# Autodesk Inventor assembly: Почти готово_CPY
(part 2 of 2)
- Жесткий:6 [WeldJoint]: Палец_CPY:1 ↔ Стопорное кольцо_CPY:2
- Жесткий:16 [WeldJoint] (-5 mm): Втулка_CPY:1 ↔ Крышка цилиндра 1_CPY:1
- Жесткий:70 [WeldJoint] (-2 mm): Фонарь_CPY:1 ↔ Крышка цилиндра 2_CPY:1
- Жесткий:79 [WeldJoint]: Крышка цилиндра 2_CPY:1 ↔ Цилиндр2_CPY:1
- Жесткий:23 [WeldJoint] (1 mm): Крышка стакана_CPY:1 ↔ Цилиндр2_CPY:1
- Жесткий:15 [WeldJoint]: Втулка_CPY:1 ↔ Цилиндр2_CPY:1
- Жесткий:18 [WeldJoint]: Цилиндр2_CPY:1 ↔ Прокладка клапана_CPY:1
- Жесткий:81 [WeldJoint] (-22 mm): Цилиндр2_CPY:1 ↔ Стакан1_CPY:1
- Жесткий:61 [WeldJoint] (2 mm): Крышка цилиндра 2_CPY:1 ↔ Уплотнительное кольцо_CPY:1
- Жесткий:69 [WeldJoint]: Фонарь_CPY:1 ↔ Уплотнение фонарь_CPY:1
- Жесткий:95 [WeldJoint]: Корпус сальника перегородка 1_CPY:1 ↔ Крышка перегородки11_CPY:1
- Жесткий:94 [WeldJoint]: Фонарь_CPY:1 ↔ Крышка перегородки11_CPY:1
- Жесткий:96 [WeldJoint]: Корпус сальника перегородка 1_CPY:1 ↔ Крышка перегородки12_CPY:1
- Жесткий:104 [WeldJoint]: Корпус маслосъемника_CPY:1 ↔ Крышка перегородки21_CPY:1
- Жесткий:98 [WeldJoint]: Фонарь_CPY:1 ↔ Крышка перегородки21_CPY:1
- Жесткий:105 [WeldJoint]: Крышка перегородки21_CPY:1 ↔ Крышка перегородки22_CPY:1
- Жесткий:97 [WeldJoint]: Фонарь_CPY:1 ↔ Придав перегородки1_CPY:1
- Жесткий:106 [WeldJoint]: Фонарь_CPY:1 ↔ Придав перегородки1_CPY:2
- Жесткий:112 [WeldJoint]: Крышка цилиндра 1_CPY:1 ↔ Шайба  ГОСТ 11371-78 25:1
- Жесткий:113 [WeldJoint] (-8.75 mm): Шпилька ГОСТ 22038-76 M24-6g×70:1 ↔ Гайка ГОСТ 15524-70 M24:1
- Жесткий:111 [WeldJoint]: Цилиндр2_CPY:1 ↔ Шпилька ГОСТ 22038-76 M24-6g×70:1
- Жесткий:114 [WeldJoint] (-8.75 mm): Шпилька ГОСТ 22038-76 M24-6g×70:2 ↔ Гайка ГОСТ 15524-70 M24:2
- Жесткий:115 [WeldJoint]: Цилиндр2_CPY:1 ↔ Прокладка клапана_CPY:2
- Жесткий:117 [WeldJoint] (-22 mm): Цилиндр2_CPY:1 ↔ Стакан1_CPY:2
- Жесткий:118 [WeldJoint] (1 mm): Цилиндр2_CPY:1 ↔ Крышка стакана_CPY:2
- Жесткий:119 [WeldJoint] (-1 mm): Цилиндр2_CPY:1 ↔ Шпилька ГОСТ 22034-76 M20-6g×50:1
- Жесткий:121 [WeldJoint] (-5.5 mm): Гайка ГОСТ 15521-70 M20:1 ↔ Шпилька ГОСТ 22034-76 M20-6g×50:1
- Жесткий:120 [WeldJoint] (-23 mm): Шпилька ГОСТ 22034-76 M20-6g×50:1 ↔ Шайба ГОСТ 10450-78 19:1
- Жесткий:122 [WeldJoint] (1 mm): Цилиндр2_CPY:1 ↔ Шпилька ГОСТ 22034-76 M20-6g×50:2
- Жесткий:124 [WeldJoint] (-6.25 mm): Шпилька ГОСТ 22034-76 M20-6g×50:2 ↔ Гайка ГОСТ 15521-70 M20:2
- Жесткий:123 [WeldJoint] (-24 mm): Шпилька ГОСТ 22034-76 M20-6g×50:2 ↔ Шайба ГОСТ 10450-78 19:2
- Жесткий:127 [WeldJoint] (-2 mm): Фонарь_CPY:1 ↔ Гайка ГОСТ 15524-70 M20:1
- Жесткий:126 [WeldJoint] (-32 mm): Шпилька ГОСТ 22038-76 M20-6g×70:1 ↔ Шайба ГОСТ 10450-78 21:1
- Жесткий:125 [WeldJoint]: Крышка цилиндра 2_CPY:1 ↔ Шпилька ГОСТ 22038-76 M20-6g×70:1
- Жесткий:130 [WeldJoint]: Крышка перегородки22_CPY:1 ↔ Шайба  ГОСТ 11371-78 13:2
- Жесткий:134 [WeldJoint]: Придав перегородки1_CPY:1 ↔ Шайба  ГОСТ 11371-78 13:4
- Жесткий:128 [WeldJoint]: Крышка перегородки12_CPY:1 ↔ Шайба  ГОСТ 11371-78 13:1
- Жесткий:135 [WeldJoint]: Шайба  ГОСТ 11371-78 13:4 ↔ Винт ГОСТ 11738-84 M 10x25:2
- Жесткий:133 [WeldJoint]: Винт ГОСТ 11738-84 M 10x25:1 ↔ Шайба  ГОСТ 11371-78 13:3
- Жесткий:132 [WeldJoint]: Придав перегородки1_CPY:2 ↔ Шайба  ГОСТ 11371-78 13:3
- Жесткий:129 [WeldJoint]: Винт ГОСТ 11738-84 M 10x35:1 ↔ Шайба  ГОСТ 11371-78 13:1
- Жесткий:131 [WeldJoint]: Винт ГОСТ 11738-84 M 10x30:1 ↔ Шайба  ГОСТ 11371-78 13:2
- Жесткий:138 [WeldJoint] (-38 mm): Шпилька ГОСТ 22038-76 M24-6g×80:1 ↔ Гайка ГОСТ 15524-70 M24:18
- Жесткий:137 [WeldJoint] (-38 mm): Шпилька ГОСТ 22038-76 M24-6g×80:1 ↔ Шайба  ГОСТ 11371-78 28:1
- Жесткий:140 [WeldJoint] (-38 mm): Шпилька ГОСТ 22038-76 M24-6g×80:2 ↔ Гайка ГОСТ 15524-70 M24:19
- Жесткий:139 [WeldJoint] (-38 mm): Шпилька ГОСТ 22038-76 M24-6g×80:2 ↔ Шайба  ГОСТ 11371-78 28:2
- Жесткий:142 [WeldJoint] (-38 mm): Шпилька ГОСТ 22038-76 M24-6g×80:3 ↔ Гайка ГОСТ 15524-70 M24:20
- Жесткий:165 [WeldJoint]: Фонарь_CPY:1 ↔ Шайба  ГОСТ 11371-78 28:3
- Жесткий:141 [WeldJoint] (-38 mm): Шпилька ГОСТ 22038-76 M24-6g×80:3 ↔ Шайба  ГОСТ 11371-78 28:3
- Жесткий:144 [WeldJoint] (-38 mm): Шпилька ГОСТ 22038-76 M24-6g×80:4 ↔ Гайка ГОСТ 15524-70 M24:21
- Жесткий:166 [WeldJoint]: Фонарь_CPY:1 ↔ Шайба  ГОСТ 11371-78 28:4
- Жесткий:143 [WeldJoint] (-38 mm): Шпилька ГОСТ 22038-76 M24-6g×80:4 ↔ Шайба  ГОСТ 11371-78 28:4
- Жесткий:146 [WeldJoint] (-38 mm): Шпилька ГОСТ 22038-76 M24-6g×80:5 ↔ Гайка ГОСТ 15524-70 M24:22
- Жесткий:164 [WeldJoint]: Фонарь_CPY:1 ↔ Шайба  ГОСТ 11371-78 28:5
- Жесткий:145 [WeldJoint] (-38 mm): Шпилька ГОСТ 22038-76 M24-6g×80:5 ↔ Шайба  ГОСТ 11371-78 28:5
- Жесткий:148 [WeldJoint] (-38 mm): Шпилька ГОСТ 22038-76 M24-6g×80:6 ↔ Гайка ГОСТ 15524-70 M24:23
- Жесткий:171 [WeldJoint]: Фонарь_CPY:1 ↔ Шайба  ГОСТ 11371-78 28:6
- Жесткий:147 [WeldJoint] (-38 mm): Шпилька ГОСТ 22038-76 M24-6g×80:6 ↔ Шайба  ГОСТ 11371-78 28:6
- Жесткий:150 [WeldJoint] (-38 mm): Шпилька ГОСТ 22038-76 M24-6g×80:7 ↔ Гайка ГОСТ 15524-70 M24:24
- Жесткий:173 [WeldJoint]: Фонарь_CPY:1 ↔ Шайба  ГОСТ 11371-78 28:7
- Жесткий:149 [WeldJoint] (-38 mm): Шпилька ГОСТ 22038-76 M24-6g×80:7 ↔ Шайба  ГОСТ 11371-78 28:7
- Жесткий:152 [WeldJoint] (-38 mm): Шпилька ГОСТ 22038-76 M24-6g×80:8 ↔ Гайка ГОСТ 15524-70 M24:25
- Жесткий:174 [WeldJoint]: Фонарь_CPY:1 ↔ Шайба  ГОСТ 11371-78 28:8
- Жесткий:151 [WeldJoint] (-38 mm): Шпилька ГОСТ 22038-76 M24-6g×80:8 ↔ Шайба  ГОСТ 11371-78 28:8
- Жесткий:154 [WeldJoint] (-38 mm): Шпилька ГОСТ 22038-76 M24-6g×80:9 ↔ Гайка ГОСТ 15524-70 M24:26
- Жесткий:172 [WeldJoint]: Фонарь_CPY:1 ↔ Шайба  ГОСТ 11371-78 28:9
- Жесткий:153 [WeldJoint] (-38 mm): Шпилька ГОСТ 22038-76 M24-6g×80:9 ↔ Шайба  ГОСТ 11371-78 28:9
- Жесткий:156 [WeldJoint] (-38 mm): Шпилька ГОСТ 22038-76 M24-6g×80:10 ↔ Гайка ГОСТ 15524-70 M24:27
- Жесткий:169 [WeldJoint]: Фонарь_CPY:1 ↔ Шайба  ГОСТ 11371-78 28:10
- Жесткий:155 [WeldJoint] (-38 mm): Шпилька ГОСТ 22038-76 M24-6g×80:10 ↔ Шайба  ГОСТ 11371-78 28:10
- Жесткий:158 [WeldJoint] (-38 mm): Шпилька ГОСТ 22038-76 M24-6g×80:11 ↔ Гайка ГОСТ 15524-70 M24:28
- Жесткий:167 [WeldJoint]: Фонарь_CPY:1 ↔ Шайба  ГОСТ 11371-78 28:11
- Жесткий:157 [WeldJoint] (-38 mm): Шпилька ГОСТ 22038-76 M24-6g×80:11 ↔ Шайба  ГОСТ 11371-78 28:11
- Жесткий:160 [WeldJoint] (-38 mm): Шпилька ГОСТ 22038-76 M24-6g×80:12 ↔ Гайка ГОСТ 15524-70 M24:29
- Жесткий:170 [WeldJoint]: Фонарь_CPY:1 ↔ Шайба  ГОСТ 11371-78 28:12
- Жесткий:159 [WeldJoint] (-38 mm): Шпилька ГОСТ 22038-76 M24-6g×80:12 ↔ Шайба  ГОСТ 11371-78 28:12
- Жесткий:162 [WeldJoint] (-38 mm): Шпилька ГОСТ 22038-76 M24-6g×80:13 ↔ Гайка ГОСТ 15524-70 M24:30
- Жесткий:168 [WeldJoint]: Фонарь_CPY:1 ↔ Шайба  ГОСТ 11371-78 28:13
- Жесткий:161 [WeldJoint] (-38 mm): Шпилька ГОСТ 22038-76 M24-6g×80:13 ↔ Шайба  ГОСТ 11371-78 28:13
- Жесткий:176 [WeldJoint] (-38 mm): Шпилька ГОСТ 22038-76 M24-6g×80:14 ↔ Гайка ГОСТ 15524-70 M24:31
- Жесткий:192 [WeldJoint]: Фонарь_CPY:1 ↔ Шайба  ГОСТ 11371-78 28:14
- Жесткий:175 [WeldJoint] (-38 mm): Шпилька ГОСТ 22038-76 M24-6g×80:14 ↔ Шайба  ГОСТ 11371-78 28:14
- Жесткий:178 [WeldJoint] (-38 mm): Шпилька ГОСТ 22038-76 M24-6g×80:15 ↔ Гайка ГОСТ 15524-70 M24:32
- Жесткий:197 [WeldJoint]: Фонарь_CPY:1 ↔ Шайба  ГОСТ 11371-78 28:15
- Жесткий:177 [WeldJoint] (-38 mm): Шпилька ГОСТ 22038-76 M24-6g×80:15 ↔ Шайба  ГОСТ 11371-78 28:15
- Жесткий:180 [WeldJoint] (-38 mm): Шпилька ГОСТ 22038-76 M24-6g×80:16 ↔ Гайка ГОСТ 15524-70 M24:33
- Жесткий:191 [WeldJoint]: Фонарь_CPY:1 ↔ Шайба  ГОСТ 11371-78 28:16
- Жесткий:179 [WeldJoint] (-38 mm): Шпилька ГОСТ 22038-76 M24-6g×80:16 ↔ Шайба  ГОСТ 11371-78 28:16
- Жесткий:184 [WeldJoint] (-38 mm): Шпилька ГОСТ 22038-76 M24-6g×80:17 ↔ Гайка ГОСТ 15524-70 M24:34
- Жесткий:196 [WeldJoint]: Фонарь_CPY:1 ↔ Шайба  ГОСТ 11371-78 28:17
- Жесткий:183 [WeldJoint] (-38 mm): Шпилька ГОСТ 22038-76 M24-6g×80:17 ↔ Шайба  ГОСТ 11371-78 28:17
- Жесткий:186 [WeldJoint] (-38 mm): Шпилька ГОСТ 22038-76 M24-6g×80:18 ↔ Гайка ГОСТ 15524-70 M24:35
- Жесткий:194 [WeldJoint]: Фонарь_CPY:1 ↔ Шайба  ГОСТ 11371-78 28:18
- Жесткий:185 [WeldJoint] (-38 mm): Шпилька ГОСТ 22038-76 M24-6g×80:18 ↔ Шайба  ГОСТ 11371-78 28:18
- Жесткий:188 [WeldJoint] (-38 mm): Шпилька ГОСТ 22038-76 M24-6g×80:19 ↔ Гайка ГОСТ 15524-70 M24:36
- Жесткий:193 [WeldJoint]: Фонарь_CPY:1 ↔ Шайба  ГОСТ 11371-78 28:19
- Жесткий:187 [WeldJoint] (-38 mm): Шпилька ГОСТ 22038-76 M24-6g×80:19 ↔ Шайба  ГОСТ 11371-78 28:19
- Жесткий:190 [WeldJoint] (-38 mm): Шпилька ГОСТ 22038-76 M24-6g×80:20 ↔ Гайка ГОСТ 15524-70 M24:37
- Жесткий:195 [WeldJoint]: Фонарь_CPY:1 ↔ Шайба  ГОСТ 11371-78 28:20
- Жесткий:189 [WeldJoint] (-38 mm): Шпилька ГОСТ 22038-76 M24-6g×80:20 ↔ Шайба  ГОСТ 11371-78 28:20
- Заподлицо:9 [Flush]: Фонарь_CPY:1 ↔ Крышка фонаря 1:1
- Заподлицо:10 [Flush]: Фонарь_CPY:1 ↔ Крышка фонаря 1:1
- Заподлицо:11 [Flush]: Фонарь_CPY:1 ↔ Крышка фонаря 2:1
- Заподлицо:12 [Flush]: Фонарь_CPY:1 ↔ Крышка фонаря 2:1
- Жесткий:395 [WeldJoint]: Крышка фонаря 1:1 ↔ Болт ГОСТ Р 50274-92 M8-6g×16-F:101
- Жесткий:396 [WeldJoint]: Крышка фонаря 1:1 ↔ Болт ГОСТ Р 50274-92 M8-6g×16-F:105
- Жесткий:397 [WeldJoint]: Крышка фонаря 1:1 ↔ Болт ГОСТ Р 50274-92 M8-6g×16-F:104
- Жесткий:398 [WeldJoint]: Крышка фонаря 1:1 ↔ Болт ГОСТ Р 50274-92 M8-6g×16-F:106
- Жесткий:399 [WeldJoint]: Крышка фонаря 1:1 ↔ Болт ГОСТ Р 50274-92 M8-6g×16-F:119
- Жесткий:400 [WeldJoint]: Крышка фонаря 1:1 ↔ Болт ГОСТ Р 50274-92 M8-6g×16-F:65
- Жесткий:401 [WeldJoint]: Крышка фонаря 1:1 ↔ Болт ГОСТ Р 50274-92 M8-6g×16-F:123
- Жесткий:402 [WeldJoint]: Крышка фонаря 1:1 ↔ Болт ГОСТ Р 50274-92 M8-6g×16-F:107
- Жесткий:403 [WeldJoint]: Крышка фонаря 1:1 ↔ Болт ГОСТ Р 50274-92 M8-6g×16-F:110
- Жесткий:404 [WeldJoint]: Крышка фонаря 1:1 ↔ Болт ГОСТ Р 50274-92 M8-6g×16-F:108
- Жесткий:405 [WeldJoint]: Крышка фонаря 1:1 ↔ Болт ГОСТ Р 50274-92 M8-6g×16-F:114
- Жесткий:406 [WeldJoint]: Крышка фонаря 1:1 ↔ Болт ГОСТ Р 50274-92 M8-6g×16-F:102
- С поворотом:3 [RevoluteJoint]: Крышка фонаря 2:1 ↔ Болт ГОСТ Р 50274-92 M8-6g×16-F:69
- С поворотом:4 [RevoluteJoint]: Крышка фонаря 2:1 ↔ Болт ГОСТ Р 50274-92 M8-6g×16-F:70
- С поворотом:5 [RevoluteJoint]: Крышка фонаря 2:1 ↔ Болт ГОСТ Р 50274-92 M8-6g×16-F:83
- Жесткий:407 [WeldJoint]: Крышка фонаря 2:1 ↔ Болт ГОСТ Р 50274-92 M8-6g×16-F:95
- Жесткий:408 [WeldJoint]: Крышка фонаря 2:1 ↔ Болт ГОСТ Р 50274-92 M8-6g×16-F:92
- Жесткий:409 [WeldJoint]: Крышка фонаря 2:1 ↔ Болт ГОСТ Р 50274-92 M8-6g×16-F:87
- Жесткий:410 [WeldJoint]: Крышка фонаря 2:1 ↔ Болт ГОСТ Р 50274-92 M8-6g×16-F:71
- Жесткий:411 [WeldJoint]: Крышка фонаря 2:1 ↔ Болт ГОСТ Р 50274-92 M8-6g×16-F:115
- Жесткий:412 [WeldJoint]: Крышка фонаря 2:1 ↔ Болт ГОСТ Р 50274-92 M8-6g×16-F:124
- Жесткий:413 [WeldJoint]: Крышка фонаря 2:1 ↔ Болт ГОСТ Р 50274-92 M8-6g×16-F:128
- Жесткий:414 [WeldJoint]: Крышка фонаря 2:1 ↔ Болт ГОСТ Р 50274-92 M8-6g×16-F:77
- Жесткий:415 [WeldJoint]: Крышка фонаря 2:1 ↔ Болт ГОСТ Р 50274-92 M8-6g×16-F:74
- Жесткий:416 [WeldJoint]: Крышка фонаря 2:1 ↔ Болт ГОСТ Р 50274-92 M8-6g×16-F:72
- Жесткий:417 [WeldJoint]: Крышка фонаря 2:1 ↔ Болт ГОСТ Р 50274-92 M8-6g×16-F:78
- Жесткий:418 [WeldJoint]: Крышка фонаря 2:1 ↔ Болт ГОСТ Р 50274-92 M8-6g×16-F:132
- Жесткий:419 [WeldJoint]: Крышка фонаря 2:1 ↔ Болт ГОСТ Р 50274-92 M8-6g×16-F:76
- Жесткий:420 [WeldJoint]: Крышка фонаря 2:1 ↔ Болт ГОСТ Р 50274-92 M8-6g×16-F:88
- Жесткий:421 [WeldJoint]: Крышка фонаря 2:1 ↔ Болт ГОСТ Р 50274-92 M8-6g×16-F:79
- Жесткий:422 [WeldJoint]: Крышка фонаря 2:1 ↔ Болт ГОСТ Р 50274-92 M8-6g×16-F:82
- Жесткий:423 [WeldJoint]: Крышка фонаря 2:1 ↔ Болт ГОСТ Р 50274-92 M8-6g×16-F:89
- Жесткий:424 [WeldJoint]: Крышка фонаря 2:1 ↔ Болт ГОСТ Р 50274-92 M8-6g×16-F:66
- Жесткий:425 [WeldJoint]: Крышка фонаря 2:1 ↔ Болт ГОСТ Р 50274-92 M8-6g×16-F:96
- Жесткий:426 [WeldJoint]: Крышка фонаря 2:1 ↔ Болт ГОСТ Р 50274-92 M8-6g×16-F:118
- Жесткий:427 [WeldJoint]: Крышка фонаря 2:1 ↔ Болт ГОСТ Р 50274-92 M8-6g×16-F:80
- Жесткий:461 [WeldJoint]: Цилиндр2_CPY:1 ↔ Деталь5_CPY:2
- Жесткий:462 [WeldJoint]: Болт ГОСТ Р 50274-92 M8-6g×16-F:175 ↔ Деталь6_CPY_MIR:1
- Жесткий:463 [WeldJoint]: Болт ГОСТ Р 50274-92 M8-6g×16-F:180 ↔ Деталь6_CPY_MIR:1
- Жесткий:464 [WeldJoint]: Болт ГОСТ Р 50274-92 M8-6g×16-F:174 ↔ Деталь6_CPY_MIR:1
- Жесткий:465 [WeldJoint]: Болт ГОСТ Р 50274-92 M8-6g×16-F:179 ↔ Деталь6_CPY_MIR:1
- Жесткий:466 [WeldJoint]: Болт ГОСТ Р 50274-92 M8-6g×16-F:178 ↔ Деталь6_CPY_MIR:1
- Жесткий:467 [WeldJoint]: Болт ГОСТ Р 50274-92 M8-6g×16-F:171 ↔ Деталь6_CPY_MIR:1
- Жесткий:468 [WeldJoint]: Болт ГОСТ Р 50274-92 M8-6g×16-F:192 ↔ Деталь6_CPY_MIR:1
- Жесткий:469 [WeldJoint]: Болт ГОСТ Р 50274-92 M8-6g×16-F:191 ↔ Деталь6_CPY_MIR:1
- Жесткий:470 [WeldJoint]: Болт ГОСТ Р 50274-92 M8-6g×16-F:190 ↔ Деталь6_CPY_MIR:1
- Жесткий:471 [WeldJoint]: Болт ГОСТ Р 50274-92 M8-6g×16-F:189 ↔ Деталь6_CPY_MIR:1
- Жесткий:472 [WeldJoint]: Болт ГОСТ Р 50274-92 M8-6g×16-F:188 ↔ Деталь6_CPY_MIR:1
- Жесткий:473 [WeldJoint]: Болт ГОСТ Р 50274-92 M8-6g×16-F:173 ↔ Деталь6_CPY_MIR:1
- Жесткий:474 [WeldJoint]: Болт ГОСТ Р 50274-92 M8-6g×16-F:172 ↔ Деталь6_CPY_MIR:1
- Жесткий:475 [WeldJoint]: Болт ГОСТ Р 50274-92 M8-6g×16-F:170 ↔ Деталь6_CPY_MIR:1
- Жесткий:476 [WeldJoint]: Болт ГОСТ Р 50274-92 M8-6g×16-F:187 ↔ Деталь6_CPY_MIR:1
- Жесткий:477 [WeldJoint]: Болт ГОСТ Р 50274-92 M8-6g×16-F:169 ↔ Деталь6_CPY_MIR:1
- Жесткий:478 [WeldJoint]: Фонарь_CPY:1 ↔ Шайба  ГОСТ 11371-78 28:1
- С поворотом:9 [RevoluteJoint] (-11 mm): Фонарь_CPY:1 ↔ Башмак_CPY:1
- Жесткий:479 [WeldJoint]: Крейцкопф_CPY:1 ↔ Прокладка крейцкопф_CPY:2
- Жесткий:480 [WeldJoint]: Фланецгайка_CPY:2 ↔ Прокладка крейцкопф_CPY:2
- Жесткий:481 [WeldJoint]: Крейцкопф_CPY:1 ↔ Шпилька ГОСТ 22038-76 M20-6g×85:3
- Жесткий:482 [WeldJoint]: Шайба  ГОСТ 11371-78 23:1 ↔ Фланецгайка_CPY:2
- Жесткий:483 [WeldJoint] (-3 mm): Шпилька ГОСТ 22038-76 M20-6g×85:3 ↔ Гайка ГОСТ 15524-70 M20:2
- Жесткий:484 [WeldJoint]: Крейцкопф_CPY:1 ↔ Шпилька ГОСТ 22038-76 M20-6g×85:2
- Жесткий:485 [WeldJoint]: Шайба  ГОСТ 11371-78 23:4 ↔ Фланецгайка_CPY:2
- Жесткий:486 [WeldJoint] (-3 mm): Шпилька ГОСТ 22038-76 M20-6g×85:2 ↔ Гайка ГОСТ 15524-70 M20:3
- [WeldJoint]: Корпус дросселя:1 ↔ Корпус сальника0:1
- [WeldJoint]: Корпус сальника 1:1 ↔ Корпус сальника0:1
- [WeldJoint]: Корпус сальника 1:1 ↔ Корпус сальника 2:1
- [WeldJoint]: Корпус сальника 2:1 ↔ Корпус сальника 3:1
- [WeldJoint]: Корпус сальника 3:1 ↔ Корпус сальника 4:1
- [WeldJoint]: Корпус сальника 4:1 ↔ В сальник:1
- [WeldJoint]: Крышка сальников:1 ↔ В сальник:1
- [WeldJoint]: Кольцо сальника:1 ↔ Пружина сальника:2
- [WeldJoint]: Кольцо сальника 2:1 ↔ Пружина сальника:3
- [WeldJoint]: Кольцо сальника 1:1 ↔ Пружина сальника:1
- [WeldJoint]: Дроссельное кольцо:1 ↔ Пружина дросселя:1
- [WeldJoint]: Кольцо сальника:2 ↔ Пружина сальника:4
- [WeldJoint]: Кольцо сальника:3 ↔ Пружина сальника:5
- [WeldJoint]: Кольцо сальника:4 ↔ Пружина сальника:6
- [WeldJoint]: Кольцо сальника:2 ↔ Кольцо сальника:3
- [WeldJoint]: Кольцо сальника:3 ↔ Кольцо сальника:4
- [WeldJoint]: Кольцо сальника 1:1 ↔ Кольцо сальника 2:1
- [WeldJoint]: Кольцо сальника 1:1 ↔ Кольцо сальника:1
- [WeldJoint]: Кольцо сальника:5 ↔ Пружина сальника:8
- [WeldJoint]: Кольцо сальника 2:2 ↔ Пружина сальника:9
- [WeldJoint]: Кольцо сальника 1:2 ↔ Пружина сальника:7
- [WeldJoint]: Кольцо сальника 1:2 ↔ Кольцо сальника 2:2
- [WeldJoint]: Кольцо сальника 1:2 ↔ Кольцо сальника:5
- [WeldJoint]: Кольцо сальника:6 ↔ Пружина сальника:10
- [WeldJoint]: Кольцо сальника:7 ↔ Пружина сальника:11
- [WeldJoint]: Кольцо сальника:8 ↔ Пружина сальника:12
- [WeldJoint]: Кольцо сальника:6 ↔ Кольцо сальника:7
- [WeldJoint]: Кольцо сальника:7 ↔ Кольцо сальника:8
- [WeldJoint]: Кольцо сальника:9 ↔ Пружина сальника:13
- [WeldJoint]: Кольцо сальника:10 ↔ Пружина сальника:14
- [WeldJoint]: Кольцо сальника:11 ↔ Пружина сальника:15
- [WeldJoint]: Кольцо сальника:9 ↔ Кольцо сальника:10
- [WeldJoint]: Кольцо сальника:10 ↔ Кольцо сальника:11
- [WeldJoint]: Кольцо сальника:12 ↔ Пружина сальника:16
- [WeldJoint]: Кольцо сальника:13 ↔ Пружина сальника:17
- [WeldJoint]: Кольцо сальника:14 ↔ Пружина сальника:18
- [WeldJoint]: Кольцо сальника:12 ↔ Кольцо сальника:13
- [WeldJoint]: Кольцо сальника:13 ↔ Кольцо сальника:14
- [WeldJoint]: Корпус дросселя:1 ↔ Дроссельное кольцо:1
- [WeldJoint]: Корпус сальника0:1 ↔ Кольцо сальника:4
- [WeldJoint]: Корпус сальника 1:1 ↔ Кольцо сальника:14
- [WeldJoint]: Корпус сальника 2:1 ↔ Кольцо сальника:8
- [WeldJoint]: Корпус сальника 3:1 ↔ Кольцо сальника:11
- [WeldJoint]: Корпус сальника 4:1 ↔ Кольцо сальника:1
- [WeldJoint]: Крышка сальников:1 ↔ Кольцо сальника:5
- Совмещение:3 [Mate] (3 mm): Крышка цилиндра 2_CPY:1 ↔ Крышка сальников:1
- [WeldJoint]: Кольцо сальника:15 ↔ Пружина сальника:20
- [WeldJoint]: Кольцо сальника 2:3 ↔ Пружина сальника:21
- [WeldJoint]: Кольцо сальника 1:3 ↔ Пружина сальника:19
- [WeldJoint]: Кольцо сальника 1:3 ↔ Кольцо сальника 2:3
- [WeldJoint]: Кольцо сальника 1:3 ↔ Кольцо сальника:15
- [WeldJoint]: Кольцо сальника:16 ↔ Пружина сальника:23
- [WeldJoint]: Кольцо сальника 2:4 ↔ Пружина сальника:24
- [WeldJoint]: Кольцо сальника 1:4 ↔ Пружина сальника:22
- [WeldJoint]: Кольцо сальника 1:4 ↔ Кольцо сальника 2:4
- [WeldJoint]: Кольцо сальника 1:4 ↔ Кольцо сальника:16
- [WeldJoint]: Кольцо сальника:18 ↔ Пружина сальника:29
- [WeldJoint]: Кольцо сальника 2:6 ↔ Пружина сальника:30
- [WeldJoint]: Кольцо сальника 1:6 ↔ Пружина сальника:28
- [WeldJoint]: Кольцо сальника 1:6 ↔ Кольцо сальника 2:6
- [WeldJoint]: Кольцо сальника 1:6 ↔ Кольцо сальника:18
- Жесткий:554 [WeldJoint]: Корпус маслосъемника_CPY:1 ↔ Кольцо сальника:16
- Жесткий:555 [WeldJoint]: Корпус сальника перегородка 1_CPY:1 ↔ Кольцо сальника:15
- Жесткий:556 [WeldJoint]: Корпус сальника перегородка 1_CPY:1 ↔ Кольцо сальника:18
- Жесткий:557 [WeldJoint] (-1 mm): Маслосъемное кольцо_CPY:1 ↔ Маслосъемная пружина_CPY:1
- Жесткий:558 [WeldJoint] (-1 mm): Маслосъемное кольцо_CPY:2 ↔ Маслосъемная пружина_CPY:2
- Жесткий:559 [WeldJoint]: Маслосъемное кольцо_CPY:1 ↔ Маслосъемное кольцо_CPY:2
- Жесткий:560 [WeldJoint]: Корпус маслосъемника_CPY:1 ↔ Маслосъемное кольцо_CPY:2
- Жесткий:561 [WeldJoint] (-22.5 mm): Цилиндр2_CPY:1 ↔ Стакан2:1
- Жесткий:562 [WeldJoint] (-22.5 mm): Цилиндр2_CPY:1 ↔ Стакан2:2
- Жесткий:563 [WeldJoint]: Стакан2:1 ↔ Клапан 2:1
- Жесткий:564 [WeldJoint]: Стакан2:2 ↔ Клапан 2:2
- Жесткий:565 [WeldJoint]: Крышка цилиндра 2_CPY:1 ↔ Шпилька ГОСТ 22038-76 M12-6g×45:1
- Жесткий:566 [WeldJoint]: Крышка сальников:1 ↔ Шайба  ГОСТ 11371-78 15:1
- Жесткий:567 [WeldJoint]: Гайка ГОСТ 15524-70 M12:1 ↔ Шайба  ГОСТ 11371-78 15:1
- Жесткий:568 [WeldJoint]: Фонарь_CPY:1 ↔ Крышка фонаря 1_MIR1:2
- Жесткий:569 [WeldJoint]: Деталь5_CPY:2 ↔ Деталь6_CPY_MIR:1
- Жесткий:570 [WeldJoint] (-44 mm): Фонарь_CPY:1 ↔ Шпилька ГОСТ 22038-76 M24-6g×80:21
- Жесткий:571 [WeldJoint]: Фонарь_CPY:1 ↔ Шайба  ГОСТ 11371-78 28:21
- Жесткий:572 [WeldJoint]: Гайка ГОСТ 15524-70 M24:53 ↔ Шайба  ГОСТ 11371-78 28:21
- Жесткий:573 [WeldJoint] (2 mm): Цилиндр2_CPY:1 ↔ Клапан0:1
- Жесткий:574 [WeldJoint] (2 mm): Цилиндр2_CPY:1 ↔ Клапан0:2
- Жесткий:575 [WeldJoint] (-3 mm): Шпилька ГОСТ 22038-76 M20-6g×85:20 ↔ Гайка ГОСТ 15524-70 M20:19
- Жесткий:576 [WeldJoint] (-3 mm): Шпилька ГОСТ 22038-76 M20-6g×85:19 ↔ Гайка ГОСТ 15524-70 M20:20
- Жесткий:578 [WeldJoint]: Цилиндр2_CPY:1 ↔ Шпилька ГОСТ 22034-76 M20-6g×50:42
- Жесткий:579 [WeldJoint]: Цилиндр2_CPY:1 ↔ Шпилька ГОСТ 22034-76 M20-6g×50:41
- Жесткий:580 [WeldJoint]: Крышка стакана_MIR_CPY:2 ↔ Шайба ГОСТ 10450-78 19:41
- Жесткий:581 [WeldJoint] (-5.25 mm): Шпилька ГОСТ 22034-76 M20-6g×50:41 ↔ Гайка ГОСТ 15521-70 M20:42
- Жесткий:582 [WeldJoint]: Крышка стакана_MIR_CPY:1 ↔ Шайба ГОСТ 10450-78 19:42
- Жесткий:583 [WeldJoint] (-5.25 mm): Шпилька ГОСТ 22034-76 M20-6g×50:42 ↔ Гайка ГОСТ 15521-70 M20:43
- Жесткий:584 [WeldJoint]: Крышка фонаря 2_MIR2:1 ↔ Болт ГОСТ Р 50274-92 M8-6g×16-F:209
- С поворотом:10 [RevoluteJoint]: Крышка фонаря 2_MIR2:1 ↔ Болт ГОСТ Р 50274-92 M8-6g×16-F:210
- С поворотом:11 [RevoluteJoint]: Крышка фонаря 2_MIR2:1 ↔ Болт ГОСТ Р 50274-92 M8-6g×16-F:211
- Жесткий:585 [WeldJoint]: Крышка фонаря 2_MIR2:1 ↔ Болт ГОСТ Р 50274-92 M8-6g×16-F:212
- Жесткий:586 [WeldJoint]: Крышка фонаря 2_MIR2:1 ↔ Болт ГОСТ Р 50274-92 M8-6g×16-F:213
- Жесткий:587 [WeldJoint]: Крышка фонаря 2_MIR2:1 ↔ Болт ГОСТ Р 50274-92 M8-6g×16-F:214
- Жесткий:588 [WeldJoint]: Крышка фонаря 2_MIR2:1 ↔ Болт ГОСТ Р 50274-92 M8-6g×16-F:215
- Жесткий:589 [WeldJoint]: Крышка фонаря 2_MIR2:1 ↔ Болт ГОСТ Р 50274-92 M8-6g×16-F:216
- Жесткий:590 [WeldJoint]: Крышка фонаря 2_MIR2:1 ↔ Болт ГОСТ Р 50274-92 M8-6g×16-F:217
- Жесткий:591 [WeldJoint]: Крышка фонаря 2_MIR2:1 ↔ Болт ГОСТ Р 50274-92 M8-6g×16-F:218
- Жесткий:592 [WeldJoint]: Крышка фонаря 2_MIR2:1 ↔ Болт ГОСТ Р 50274-92 M8-6g×16-F:219
- Жесткий:593 [WeldJoint]: Крышка фонаря 2_MIR2:1 ↔ Болт ГОСТ Р 50274-92 M8-6g×16-F:220
- С поворотом:12 [RevoluteJoint]: Крышка фонаря 2_MIR2:1 ↔ Болт ГОСТ Р 50274-92 M8-6g×16-F:221
- Жесткий:594 [WeldJoint]: Крышка фонаря 2_MIR2:1 ↔ Болт ГОСТ Р 50274-92 M8-6g×16-F:222
- Жесткий:595 [WeldJoint]: Крышка фонаря 2_MIR2:1 ↔ Болт ГОСТ Р 50274-92 M8-6g×16-F:223
- Жесткий:596 [WeldJoint]: Крышка фонаря 2_MIR2:1 ↔ Болт ГОСТ Р 50274-92 M8-6g×16-F:224
- Жесткий:597 [WeldJoint]: Крышка фонаря 2_MIR2:1 ↔ Болт ГОСТ Р 50274-92 M8-6g×16-F:225
- Жесткий:598 [WeldJoint]: Крышка фонаря 2_MIR2:1 ↔ Болт ГОСТ Р 50274-92 M8-6g×16-F:226
- Жесткий:599 [WeldJoint]: Крышка фонаря 2_MIR2:1 ↔ Болт ГОСТ Р 50274-92 M8-6g×16-F:227
- Жесткий:600 [WeldJoint]: Крышка фонаря 2_MIR2:1 ↔ Болт ГОСТ Р 50274-92 M8-6g×16-F:228
- Жесткий:601 [WeldJoint]: Крышка фонаря 2_MIR2:1 ↔ Болт ГОСТ Р 50274-92 M8-6g×16-F:229
- Жесткий:602 [WeldJoint]: Крышка фонаря 2_MIR2:1 ↔ Болт ГОСТ Р 50274-92 M8-6g×16-F:230
- Жесткий:603 [WeldJoint]: Крышка фонаря 2_MIR2:1 ↔ Болт ГОСТ Р 50274-92 M8-6g×16-F:231
- Жесткий:604 [WeldJoint]: Крышка фонаря 2_MIR2:1 ↔ Болт ГОСТ Р 50274-92 M8-6g×16-F:232
- [WeldJoint]: Гайка шток-поршень_CPY:2 ↔ Кольцо поршень-шток верх_CPY:2
- [WeldJoint]: Верхняя часть поршня_CPY:2 ↔ Кольцо поршень-шток верх_CPY:2
- [WeldJoint]: Верхняя часть поршня_CPY:2 ↔ Кольцо поршня_CPY:4
- [WeldJoint]: Кольцо поршень-шток низ_CPY:2 ↔ Нижняя часть поршня_CPY:2
- [WeldJoint]: Верхняя часть поршня_CPY:2 ↔ Нижняя часть поршня_CPY:2
- [WeldJoint]: Нижняя часть поршня_CPY:2 ↔ Опорное кольцо_CPY:3
- [WeldJoint]: Нижняя часть поршня_CPY:2 ↔ Кольцо поршня_CPY:5
- [WeldJoint]: Нижняя часть поршня_CPY:2 ↔ Кольцо поршня_CPY:6
- [WeldJoint]: Верхняя часть поршня_CPY:2 ↔ Опорное кольцо_CPY:4
- [WeldJoint] (4.75 mm): Гайка шток-поршень_CPY:2 ↔ Шток_CPY:2
## Named parameters: d653_d28_d11_d7 = 0 mm, d654_d29_d12_d7 = 0 mm, d655_d30_d13_d7 = 0 mm, d656_d31_d14 = 0 mm, d657_d32_d15 = 0 mm, d658_d33_d11_d7 = 0 mm, d659_d34_d12_d7 = 0 mm, d660_d35_d13_d7 = 0 mm, d661_d36_d14 = 0 mm, d662_d37_d15 = 0 mm, d663_d38 = 0 mm, d664_d39 = 0 mm, d665_d40 = 0 mm, d666_d41 = 0 mm, d667_d42 = 0 mm, d668_d43 = 0 mm, d669_d44 = 0 mm, d670_d7 = 0 mm, d671_d8 = 0 mm, d672_d9 = 0 mm, d673_d10 = 0 mm, d674_d11_d7 = 0 mm, d675_d12_d7 = 0 mm, d676_d13_d7 = 0 mm, d677_d14 = 0 mm, d678_d15 = 0 mm, d679_d16 = 0 mm, d680_d17 = 0 mm, d681_d18_d7 = 0 mm, d682_d19_d8 = 0 mm, d683_d20_d9 = 0 mm, d684_d21_d16 = 0 mm, d685_d22_d17 = 0 mm, d686_d23_d11_d7 = 0 mm, d687_d24_d12_d7 = 0 mm, d688_d25_d13_d7 = 0 mm, d689_d26_d14 = 0 mm, d690_d27_d15 = 0 mm, d644_d679_d16 = 0 mm, d645_d680_d17 = 0 mm, d646_d681_d18_d7 = 0 mm, d647_d682_d19_d8 = 0 mm, d648_d683_d20_d9 = 0 mm, d649_d684_d21_d16 = 0 mm, d650_d685_d22_d17 = 0 mm, d651_d670_d7 = 0 mm, d652_d671_d8 = 0 mm, d653_d672_d9 = 0 mm, d656_d646_d681_d18_d7 = 0 mm, d657_d647_d682_d19_d8 = 0 mm, d658_d648_d683_d20_d9 = 0 mm, d659_d649_d684_d21_d16 = 0 mm, d660_d650_d685_d22_d17 = 0 mm, d734_d20 = 0 mm, d735_d21 = 0 mm, d736_d22 = 0 mm, d737_d27 = 0 mm, d738_d28 = 0 mm, d739_d29 = 0 mm, d740_d119 = 4.75 mm, d741_d34 = 0 mm, d742_d37 = 0 mm, d743_d41 = 0 mm
